# Autodesk Inventor assembly: Prototipo 2
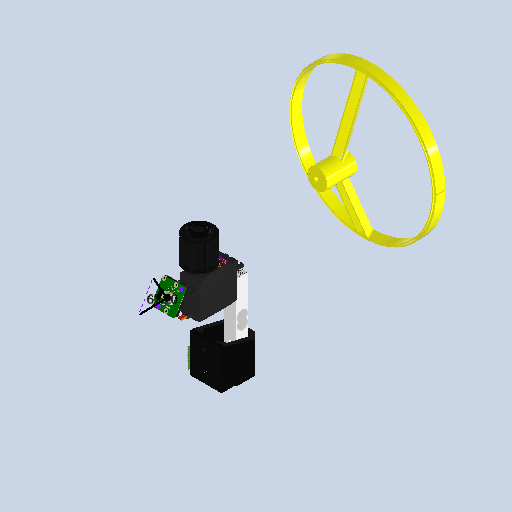
[picture p0: Inventor's stored thumbnail of the model, 512x512]
Saved by Autodesk Inventor 2023 (Build 270158000, 158)
## iProperties
Created: 2021-02-18
Part Number: Prototipo 2
Document SubType Name: Assembly
Designer: juanp
Author: juanp
## Documents named in this file (13)
- C:\Users\juanp\OneDrive - Universidad de los andes\Uniandes\Robocol\EVA\V3 (Actual)\Dispensador\Dispensador V3.iam
- C:\Users\juanp\OneDrive - Universidad de los andes\Uniandes\Robocol\EVA\Recursos\Servo MG996R\Servo Motor MG996R.iam
- C:\Users\juanp\OneDrive - Universidad de los andes\Uniandes\Robocol\EVA\V3 (Actual)\Dispensador\attachmentcustom V2.ipt
- C:\Users\juanp\OneDrive - Universidad de los andes\Uniandes\Robocol\EVA\V3 (Actual)\Dispensador\Valvula V2.ipt
- C:\Users\juanp\OneDrive - Universidad de los andes\Uniandes\Robocol\EVA\V3 (Actual)\Dispensador\Retenedor.ipt
- C:\Users\juanp\OneDrive - Universidad de los andes\Uniandes\Robocol\EVA\V3 (Actual)\Dispensador\Carcasa V2.ipt
- C:\Users\juanp\OneDrive - Universidad de los andes\Uniandes\Robocol\EVA\Recursos\Celda de Carga\CELDA DE PRESION ARDUINO.ipt
- C:\Users\juanp\OneDrive - Universidad de los andes\Uniandes\Robocol\EVA\V3 (Actual)\Dispensador\Soporte Actuador V2.ipt
- C:\Users\juanp\OneDrive - Universidad de los andes\Uniandes\Robocol\EVA\V3 (Actual)\Camara\Case.ipt
- C:\Users\juanp\OneDrive - Universidad de los andes\Uniandes\Robocol\EVA\Recursos\Pi Camera\RspCameraMia.iam
- C:\Users\juanp\OneDrive - Universidad de los andes\Uniandes\Robocol\EVA\V3 (Actual)\Dispensador\Arandela HX711.ipt
- C:\Users\juanp\OneDrive - Universidad de los andes\Uniandes\Robocol\EVA\Recursos\HX711\Hx711 Full.ipt
- C:\Users\juanp\OneDrive - Universidad de los andes\Uniandes\Robocol\EVA\Recursos\Servo MG996R\attachment disp.ipt
## Components (16 placed, 12 different names)
1. Servo Motor MG996R:1 [sub-assembly] — Mate:1, Mate:2, Flush:1, Mate:11, Mate:43, Mate:44, Mate:51, Mate:52
2. attachmentcustom V2:1 — Mate:42, Flush:8, Mate:50, Flush:9
3. Valvula V2:1 — Mate:7, Mate:8, Mate:48, Mate:49, Mate:50
4. Retenedor:1 — Mate:7, Mate:48, Flush:9
5. Retenedor:2 — Mate:8, Mate:49
6. Carcasa V2:1 — Mate:11, Mate:23, Mate:24, Mate:25, Mate:29, Flush:4, Flush:5, Mate:42, Flush:8, Mate:43, Mate:44
7. CELDA DE PRESION ARDUINO:1 — Mate:23, Mate:24, Mate:25, Mate:26, Mate:27, Mate:28
8. Soporte Actuador V2:1 — Mate:26, Mate:27, Mate:28, Mate:53, Mate:54, Mate:55, Mate:56
9. Case:1 — Mate:29, Mate:30, Mate:31, Mate:32, Flush:5
10. RspCameraMia:1 [sub-assembly] — Mate:30, Mate:31, Mate:32, Flush:4
11. Arandela HX711:1 — Mate:53, Mate:55, Mate:58, Mate:59
12. Arandela HX711:2 — Mate:61, Mate:62
13. Arandela HX711:3 — Mate:60, Mate:63
14. Arandela HX711:4 — Mate:54, Mate:56, Mate:57
15. Hx711 Full:1 — Mate:57, Mate:58, Mate:59, Mate:60, Mate:61, Mate:62, Mate:63
16. attachment disp:1 — Mate:51, Mate:52
## Relationships (39: Mate 34, Flush 5)
- Mate:1: Servo Motor MG996R:1
- Mate:2: Servo Motor MG996R:1
- Flush:1: Servo Motor MG996R:1
- Mate:7: Valvula V2:1 ↔ Retenedor:1
- Mate:8: Valvula V2:1 ↔ Retenedor:2
- Mate:11: Servo Motor MG996R:1 ↔ Carcasa V2:1
- Mate:23: Carcasa V2:1 ↔ CELDA DE PRESION ARDUINO:1
- Mate:24: Carcasa V2:1 ↔ CELDA DE PRESION ARDUINO:1
- Mate:25: Carcasa V2:1 ↔ CELDA DE PRESION ARDUINO:1
- Mate:26: CELDA DE PRESION ARDUINO:1 ↔ Soporte Actuador V2:1
- Mate:27: CELDA DE PRESION ARDUINO:1 ↔ Soporte Actuador V2:1
- Mate:28: CELDA DE PRESION ARDUINO:1 ↔ Soporte Actuador V2:1
- Mate:29: Carcasa V2:1 ↔ Case:1
- Mate:30: Case:1 ↔ RspCameraMia:1
- Mate:31: Case:1 ↔ RspCameraMia:1
- Mate:32: Case:1 ↔ RspCameraMia:1
- Flush:4: Carcasa V2:1 ↔ RspCameraMia:1
- Flush:5: Carcasa V2:1 ↔ Case:1
- Mate:42: attachmentcustom V2:1 ↔ Carcasa V2:1
- Flush:8: attachmentcustom V2:1 ↔ Carcasa V2:1
- Mate:43: Servo Motor MG996R:1 ↔ Carcasa V2:1
- Mate:44: Servo Motor MG996R:1 ↔ Carcasa V2:1
- Mate:48: Valvula V2:1 ↔ Retenedor:1
- Mate:49: Valvula V2:1 ↔ Retenedor:2
- Mate:50: attachmentcustom V2:1 ↔ Valvula V2:1
- Mate:51: Servo Motor MG996R:1 ↔ attachment disp:1
- Mate:52: Servo Motor MG996R:1 ↔ attachment disp:1
- Mate:53: Soporte Actuador V2:1 ↔ Arandela HX711:1
- Mate:54: Soporte Actuador V2:1 ↔ Arandela HX711:4
- Mate:55: Soporte Actuador V2:1 ↔ Arandela HX711:1
- Mate:56: Soporte Actuador V2:1 ↔ Arandela HX711:4
- Mate:57: Arandela HX711:4 ↔ Hx711 Full:1
- Mate:58: Arandela HX711:1 ↔ Hx711 Full:1
- Mate:59: Arandela HX711:1 ↔ Hx711 Full:1
- Mate:60: Arandela HX711:3 ↔ Hx711 Full:1
- Mate:61: Arandela HX711:2 ↔ Hx711 Full:1
- Mate:62: Arandela HX711:2 ↔ Hx711 Full:1
- Mate:63: Arandela HX711:3 ↔ Hx711 Full:1
- Flush:9 (3.25 mm): attachmentcustom V2:1 ↔ Retenedor:1
